# Autodesk Inventor assembly: OCT_Probe_Asm_03142013
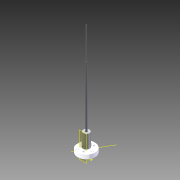
[picture p0: Inventor's stored thumbnail of the model, 180x180]
Saved by Autodesk Inventor 2011 SP2 (Build 150309200, 309)
## iProperties
Created: 2012-04-17
Part Number: OCT_Probe_Asm_03142013
Document SubType Name: Assembly
Designer: sungwook
Author: sungwook
## Documents named in this file (4)
- C:\Users\sungwook\Documents\Inventor\Micron22_top_adj_02082013\OCT Probes\OCT_Probe_Asm_03142013.iam
- C:\Users\sungwook\Documents\Inventor\Micron22_top_adj_02082013\Parts\Tool\Tool_Mount_Luer_Adapter.ipt
- C:\Users\sungwook\Documents\Inventor\Micron22_top_adj_02082013\Parts\Tool\Tool Mount_Rev.ipt
- C:\Users\sungwook\Documents\Inventor\Micron22_top_adj_02082013\OCT Probes\OCT_Probe_Asm_wo_luer.iam
## Components (3 placed, 3 different names)
1. Tool_Mount_Luer_Adapter:1 — Mate:8, Mate:12, Mate:13, Flush:8, Mate:14
2. Tool Mount_Rev:1 — Mate:12, Mate:13, Angle:1
3. OCT_Probe_Asm_wo_luer:1 [sub-assembly] — Flush:8, Mate:14
## Relationships (6: Mate 4, Angle 1, Flush 1)
- Mate:8: Tool_Mount_Luer_Adapter:1
- Mate:12: Tool_Mount_Luer_Adapter:1 ↔ Tool Mount_Rev:1
- Mate:13: Tool_Mount_Luer_Adapter:1 ↔ Tool Mount_Rev:1
- Angle:1 (180 deg): Tool Mount_Rev:1
- Flush:8: Tool_Mount_Luer_Adapter:1 ↔ OCT_Probe_Asm_wo_luer:1
- Mate:14: Tool_Mount_Luer_Adapter:1 ↔ OCT_Probe_Asm_wo_luer:1
